# Autodesk Inventor assembly: offset_gear2
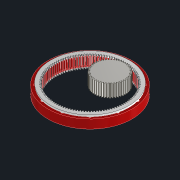
[picture p0: Inventor's stored thumbnail of the model, 180x180]
Saved by Autodesk Inventor 2021 (Build 250183000, 183)
## iProperties
Created: 2021-08-19
Part Number: offset_gear2
Document SubType Name: Assembly
Designer: yuta0
Author: yuta0
## Documents named in this file (3)
- C:\Users\yuta0\Documents\GitHub\catchrobo_hardware\assy-robot\offset_gear2.iam
- C:\Users\yuta0\Documents\GitHub\catchrobo_hardware\assy-robot\offset_gear2\デザイン アクセラレータ\平歯車2.iam
- C:\Users\yuta0\Documents\GitHub\catchrobo_hardware\assy-robot\base33.ipt
## Components (2 placed, 2 different names)
1. 平歯車:1 [sub-assembly] — メイト:1
2. base33:1 — メイト:1
## Relationships (1: Mate 1)
- メイト:1 [Mate]: 平歯車:1 ↔ base33:1
